# Autodesk Inventor assembly: Gripper
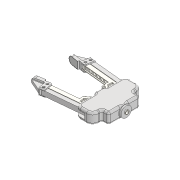
[picture p0: Inventor's stored thumbnail of the model, 180x180]
Saved by Autodesk Inventor 2020.3 (Build 243373010, 373A)
## iProperties
Created: 2021-05-15
Part Number: Gripper
Document SubType Name: Assembly
Designer: marti
Author: marti
## Documents named in this file (3)
- C:\Users\marti\Documents\Inventor\RobotManipulateArm\17.4.2021 - Complete new IDEA\Gripper.iam
- C:\Users\marti\Documents\Inventor\RobotManipulateArm\17.4.2021 - Complete new IDEA\Worm shaft tilting head - gripper.iam
- C:\Users\marti\Documents\Inventor\RobotManipulateArm\17.4.2021 - Complete new IDEA\Housing of gripper.ipt
## Components (2 placed, 2 different names)
1. Worm shaft tilting head - gripper:1 [sub-assembly] — Mate:1, Flush:1, Flush:2
2. Housing of gripper:1 — Mate:1, Flush:1, Flush:2
## Relationships (3: Flush 2, Mate 1)
- Mate:1 (1.25 mm): Worm shaft tilting head - gripper:1 ↔ Housing of gripper:1
- Flush:1: Worm shaft tilting head - gripper:1 ↔ Housing of gripper:1
- Flush:2: Worm shaft tilting head - gripper:1 ↔ Housing of gripper:1
